# Autodesk Inventor assembly: BoltWasher5x10
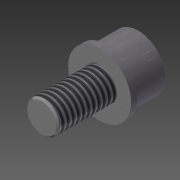
[picture p0: Inventor's stored thumbnail of the model, 180x180]
Saved by Autodesk Inventor 2015 SP1 (Build 190203100, 203)
## iProperties
Category: Hardware
Created: 2014-08-08
Part Number: BoltWasher5x10
Document SubType Name: Assembly
Designer: t_clevj
Vendor: Misumi
Author: Jack
Title: Bolt + Washer SHCS 5 x 10
## Documents named in this file (3)
- C:\Users\Jack\ownCloud\Projects\CoreXY\InventorModel\Hardware\BoltWashers\BoltWasher5\BoltWasher5x10.iam
- C:\Users\Jack\ownCloud\Projects\CoreXY\InventorModel\Hardware\Bolts\SHCS\SHCS5\SHCS5x10.ipt
- C:\Users\Jack\ownCloud\Projects\CoreXY\InventorModel\Hardware\Wahsers\M5Washer.ipt
## Components (2 placed, 2 different names)
1. SHCS5x10:1 — Mate:1, Mate:2
2. M5Washer:1 — Mate:1, Mate:2
## Relationships (2: Mate 2)
- Mate:1: SHCS5x10:1 ↔ M5Washer:1
- Mate:2: SHCS5x10:1 ↔ M5Washer:1
